# Autodesk Inventor assembly: robot_simu
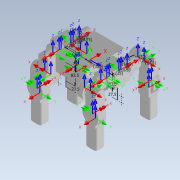
[picture p0: Inventor's stored thumbnail of the model, 180x180]
Saved by Autodesk Inventor 2020 (Build 240168000, 168)
## iProperties
Created: 2021-01-12
Part Number: robot_simu
Document SubType Name: Assembly
Designer: DELL
Author: DELL
## Documents named in this file (13)
- F:\SoftRobot2.0\FlexipodHardware2.0\FlexipodHardware\Flexipod2.0\Cadquery_module\v3.0\robot_simu.iam
- F:\SoftRobot2.0\FlexipodHardware2.0\FlexipodHardware\Flexipod2.0\Cadquery_module\v3.0\body_motor_fix_board_left.ipt
- F:\SoftRobot2.0\FlexipodHardware2.0\FlexipodHardware\Flexipod2.0\Cadquery_module\v3.0\body_motor_fix_board_right.ipt
- F:\SoftRobot2.0\FlexipodHardware2.0\FlexipodHardware\Flexipod2.0\Cadquery_module\v3.0\motor.ipt
- F:\SoftRobot2.0\FlexipodHardware2.0\FlexipodHardware\Flexipod2.0\Cadquery_module\v3.0\hip_front_left.ipt
- F:\SoftRobot2.0\FlexipodHardware2.0\FlexipodHardware\Flexipod2.0\Cadquery_module\v3.0\hip_front_right.ipt
- F:\SoftRobot2.0\FlexipodHardware2.0\FlexipodHardware\Flexipod2.0\Cadquery_module\v3.0\left_thigh.ipt
- F:\SoftRobot2.0\FlexipodHardware2.0\FlexipodHardware\Flexipod2.0\Cadquery_module\v3.0\right_thigh.ipt
- F:\SoftRobot2.0\FlexipodHardware2.0\FlexipodHardware\Flexipod2.0\Cadquery_module\v3.0\shank_board.ipt
- F:\SoftRobot2.0\FlexipodHardware2.0\FlexipodHardware\Flexipod2.0\Cadquery_module\v3.0\shank.ipt
- F:\SoftRobot2.0\FlexipodHardware2.0\FlexipodHardware\Flexipod2.0\Cadquery_module\v3.0\hip_back_left.ipt
- F:\SoftRobot2.0\FlexipodHardware2.0\FlexipodHardware\Flexipod2.0\Cadquery_module\v3.0\hip_back_right.ipt
- F:\SoftRobot2.0\FlexipodHardware2.0\FlexipodHardware\Flexipod2.0\Cadquery_module\v3.0\body_2.ipt
## Components (33 placed, 12 different names)
1. body_motor_fix_board_left:1 — Mate:6, Mate:71, Flush:6, Flush:7
2. body_motor_fix_board_left:2 — Mate:18, Mate:73, Flush:9, Flush:10, Flush:81
3. body_motor_fix_board_right:1 — Mate:11, Mate:72, Flush:8, Flush:11, Flush:82
4. body_motor_fix_board_right:2 — Mate:8, Mate:70, Flush:4, Flush:5
5. motor:1 — Mate:6, Mate:14, Mate:15, Mate:74, Angle:40
6. motor:2 — Mate:8, Mate:12, Mate:13, Mate:78, Angle:33
7. motor:3 — Mate:18, Mate:39, Mate:40, Flush:81, Mate:81
8. motor:4 — Mate:11, Mate:37, Mate:38, Flush:82, Mate:84
9. hip_front_left:1 — Mate:14, Mate:15, Mate:16, Mate:17, Angle:7, Mate:61
10. hip_front_right:1 — Mate:12, Mate:13, Mate:19, Mate:20
11. motor:5 — Mate:16, Mate:17, Angle:7, Mate:21, Mate:22
12. motor:6 — Mate:19, Mate:20, Mate:23, Mate:24, Flush:12
13. left_thigh:1 — Mate:21, Mate:22, Mate:27, Mate:28, Angle:12, Angle:13, Angle:29, Angle:30
14. right_thigh:1 — Mate:23, Mate:24, Mate:25, Mate:26, Angle:11, Angle:14, Angle:31, Angle:32, Flush:12
15. motor:7 — Mate:25, Mate:26, Angle:11, Mate:32, Mate:77
16. motor:8 — Mate:27, Mate:28, Angle:12, Mate:30, Mate:75
17. shank_board:1 — Mate:32, Angle:14, Angle:16, Mate:63, Mate:77, Mate:79
18. shank_board:2 — Mate:30, Angle:13, Mate:36, Angle:15, Mate:75, Mate:76
19. shank:1 — Mate:36, Angle:15, Mate:76
20. shank:2 — Angle:16, Mate:63, Mate:79
21. hip_back_left:1 — Mate:39, Mate:40, Mate:43, Mate:44, Angle:34, Angle:36
22. hip_back_right:1 — Mate:37, Mate:38, Mate:41, Mate:42, Angle:37, Angle:38, Angle:39
23. motor:9 — Mate:41, Mate:42, Mate:45, Mate:46, Angle:38
24. motor:10 — Mate:43, Mate:44, Mate:47, Mate:48, Angle:35, Angle:36
25. left_thigh:2 — Mate:47, Mate:48, Mate:51, Mate:52, Angle:24, Angle:26, Angle:28, Angle:35
26. right_thigh:2 — Mate:45, Mate:46, Mate:49, Mate:50, Angle:23, Angle:25, Angle:27, Angle:39
27. motor:11 — Mate:49, Mate:50, Angle:23, Mate:55, Mate:85
28. motor:12 — Mate:51, Mate:52, Angle:24, Mate:56, Mate:82
29. shank_board:3 — Mate:56, Angle:26, Mate:64, Mate:82, Mate:83
30. shank_board:4 — Mate:55, Angle:25, Mate:65, Mate:85, Mate:86
31. shank:3 — Angle:27, Mate:65, Mate:86
32. shank:4 — Angle:28, Mate:64, Mate:83
33. body_2:1 — Flush:1, Flush:2, Flush:3, Mate:70, Flush:4, Flush:5, Mate:71, Flush:6, Flush:7, Mate:72, Flush:8, Mate:73, Flush:9, Flush:10, Flush:11, Mate:74, Angle:29, Mate:78, Angle:30, Angle:31, Angle:32, Angle:33, Mate:81, Angle:34, Mate:84, Angle:37, Angle:40
## Relationships (101: Mate 62, Angle 25, Flush 14)
- Mate:6: body_motor_fix_board_left:1 ↔ motor:1
- Mate:8: body_motor_fix_board_right:2 ↔ motor:2
- Mate:11: body_motor_fix_board_right:1 ↔ motor:4
- Mate:12: motor:2 ↔ hip_front_right:1
- Mate:13: motor:2 ↔ hip_front_right:1
- Mate:14: motor:1 ↔ hip_front_left:1
- Mate:15: motor:1 ↔ hip_front_left:1
- Mate:16: hip_front_left:1 ↔ motor:5
- Mate:17: hip_front_left:1 ↔ motor:5
- Angle:7 (0 deg): hip_front_left:1 ↔ motor:5
- Mate:18: body_motor_fix_board_left:2 ↔ motor:3
- Mate:19: hip_front_right:1 ↔ motor:6
- Mate:20: hip_front_right:1 ↔ motor:6
- Mate:21: motor:5 ↔ left_thigh:1
- Mate:22: motor:5 ↔ left_thigh:1
- Mate:23: motor:6 ↔ right_thigh:1
- Mate:24: motor:6 ↔ right_thigh:1
- Mate:25: right_thigh:1 ↔ motor:7
- Mate:26: right_thigh:1 ↔ motor:7
- Angle:11 (180 deg): right_thigh:1 ↔ motor:7
- Mate:27: left_thigh:1 ↔ motor:8
- Mate:28: left_thigh:1 ↔ motor:8
- Angle:12 (0 deg): left_thigh:1 ↔ motor:8
- Mate:30: motor:8 ↔ shank_board:2
- Angle:13 (0 deg): left_thigh:1 ↔ shank_board:2
- Mate:32: motor:7 ↔ shank_board:1
- Angle:14 (0 deg): right_thigh:1 ↔ shank_board:1
- Mate:36: shank_board:2 ↔ shank:1
- Angle:15 (180 deg): shank_board:2 ↔ shank:1
- Angle:16 (0 deg): shank_board:1 ↔ shank:2
- Mate:37: motor:4 ↔ hip_back_right:1
- Mate:38: motor:4 ↔ hip_back_right:1
- Mate:39: motor:3 ↔ hip_back_left:1
- Mate:40: motor:3 ↔ hip_back_left:1
- Mate:41: hip_back_right:1 ↔ motor:9
- Mate:42: hip_back_right:1 ↔ motor:9
- Mate:43: hip_back_left:1 ↔ motor:10
- Mate:44: hip_back_left:1 ↔ motor:10
- Mate:45: motor:9 ↔ right_thigh:2
- Mate:46: motor:9 ↔ right_thigh:2
- Mate:47: motor:10 ↔ left_thigh:2
- Mate:48: motor:10 ↔ left_thigh:2
- Mate:49: right_thigh:2 ↔ motor:11
- Mate:50: right_thigh:2 ↔ motor:11
- Mate:51: left_thigh:2 ↔ motor:12
- Mate:52: left_thigh:2 ↔ motor:12
- Angle:23 (180 deg): right_thigh:2 ↔ motor:11
- Angle:24 (0 deg): left_thigh:2 ↔ motor:12
- Mate:55: motor:11 ↔ shank_board:4
- Mate:56: motor:12 ↔ shank_board:3
- Angle:25 (0 deg): right_thigh:2 ↔ shank_board:4
- Angle:26 (0 deg): left_thigh:2 ↔ shank_board:3
- Angle:27 (0 deg): right_thigh:2 ↔ shank:3
- Angle:28 (180 deg): left_thigh:2 ↔ shank:4
- Mate:61: hip_front_left:1
- Mate:62
- Mate:63: shank_board:1 ↔ shank:2
- Mate:64: shank_board:3 ↔ shank:4
- Mate:65: shank_board:4 ↔ shank:3
- Flush:1: body_2:1
- Flush:2: body_2:1
- Flush:3: body_2:1
- Mate:70: body_motor_fix_board_right:2 ↔ body_2:1
- Flush:4: body_motor_fix_board_right:2 ↔ body_2:1
- Flush:5: body_motor_fix_board_right:2 ↔ body_2:1
- Mate:71: body_motor_fix_board_left:1 ↔ body_2:1
- Flush:6: body_motor_fix_board_left:1 ↔ body_2:1
- Flush:7: body_motor_fix_board_left:1 ↔ body_2:1
- Mate:72: body_motor_fix_board_right:1 ↔ body_2:1
- Flush:8: body_motor_fix_board_right:1 ↔ body_2:1
- Mate:73: body_motor_fix_board_left:2 ↔ body_2:1
- Flush:9: body_motor_fix_board_left:2 ↔ body_2:1
- Flush:10: body_motor_fix_board_left:2 ↔ body_2:1
- Flush:11: body_motor_fix_board_right:1 ↔ body_2:1
- Mate:74: motor:1 ↔ body_2:1
- Mate:75: motor:8 ↔ shank_board:2
- Mate:76: shank_board:2 ↔ shank:1
- Angle:29 (0 deg): left_thigh:1 ↔ body_2:1
- Mate:77: motor:7 ↔ shank_board:1
- Mate:78: motor:2 ↔ body_2:1
- Mate:79: shank_board:1 ↔ shank:2
- Angle:30 (0 deg): left_thigh:1 ↔ body_2:1
- Angle:31 (0 deg): right_thigh:1 ↔ body_2:1
- Angle:32 (0 deg): right_thigh:1 ↔ body_2:1
- Flush:12: motor:6 ↔ right_thigh:1
- Angle:33 (0 deg): motor:2 ↔ body_2:1
- Flush:81: body_motor_fix_board_left:2 ↔ motor:3
- Mate:81: motor:3 ↔ body_2:1
- Angle:34 (0 deg): hip_back_left:1 ↔ body_2:1
- Angle:35 (0 deg): motor:10 ↔ left_thigh:2
- Angle:36 (0 deg): hip_back_left:1 ↔ motor:10
- Mate:82: motor:12 ↔ shank_board:3
- Mate:83: shank_board:3 ↔ shank:4
- Flush:82: body_motor_fix_board_right:1 ↔ motor:4
- Mate:84: motor:4 ↔ body_2:1
- Angle:37 (0 deg): hip_back_right:1 ↔ body_2:1
- Angle:38 (180 deg): hip_back_right:1 ↔ motor:9
- Angle:39 (0 deg): hip_back_right:1 ↔ right_thigh:2
- Mate:85: motor:11 ↔ shank_board:4
- Mate:86: shank_board:4 ↔ shank:3
- Angle:40 (180 deg): motor:1 ↔ body_2:1
